# Autodesk Inventor assembly: ClawLauncher
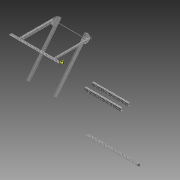
[picture p0: Inventor's stored thumbnail of the model, 180x180]
Saved by Autodesk Inventor 2015 (Build 190159000, 159)
## iProperties
Created: 2016-09-16
Part Number: ClawLauncher
Document SubType Name: Assembly
Designer: wangl
Author: wangl
## Documents named in this file (14)
- M:\StarStuck Prototypes\Prototypes\ClawLauncher.iam
- M:\StarStuck Prototypes\Imported Components\C-Channel 1x2x1x35\C-Channel 1x2x1x35 2.0.ipt
- M:\StarStuck Prototypes\Imported Components\C- Channel 1x2x1x25 2.0\C- Channel 1x2x1x25 2.0.ipt
- M:\StarStuck Prototypes\Imported Components\Chasis Rail 2x1x25\Chasis Rail 2x1x25.ipt
- M:\StarStuck Prototypes\Imported Components\Angle 2x2x35\Angle 2x2x35.ipt
- M:\StarStuck Prototypes\Imported Components\Large Screw .500In\Large Screw .500In.ipt
- M:\StarStuck Prototypes\Imported Components\Flat Bearing\Flat Bearing.ipt
- M:\StarStuck Prototypes\Imported Components\Large Screw .25In\Large Screw .25In.ipt
- M:\StarStuck Prototypes\Imported Components\Regular Nut\Regular Nut.ipt
- M:\StarStuck Prototypes\Imported Components\Axle 12in\Axle 12in.ipt
- M:\StarStuck Prototypes\Imported Components\Shaft Collar\Shaft Collar.ipt
- M:\StarStuck Prototypes\Imported Components\60T HS Gear\60T HS Gear.ipt
- M:\StarStuck Prototypes\Imported Components\HS Gear Metal Insert\HS Gear Metal Insert.ipt
- M:\StarStuck Prototypes\Imported Components\Large 1.00in Screw\Large 1.00in Screw.ipt
## Components (39 placed, 13 different names)
1. C-Channel 1x2x1x35 2.0:1 — Mate:44, Tangent:29, Tangent:30, Tangent:32, Tangent:37
2. C- Channel 1x2x1x25 2.0:1
3. C- Channel 1x2x1x25 2.0:2
4. Chasis Rail 2x1x25:1 — Flush:4, Mate:4, Flush:6, Mate:13, Tangent:13, Tangent:14, Tangent:15, Tangent:16, Mate:16, Mate:17, Mate:23, Mate:24, Tangent:26
5. Chasis Rail 2x1x25:2 — Mate:3, Flush:3, Flush:5, Mate:5, Mate:6, Mate:7, Tangent:7, Tangent:8, Tangent:9, Tangent:10, Mate:14, Mate:15
6. C-Channel 1x2x1x35 2.0:2 — Mate:43, Tangent:33, Tangent:34, Tangent:35, Tangent:36
7. Angle 2x2x35:1
8. Angle 2x2x35:2 — Mate:3, Flush:3, Flush:4, Mate:4, Flush:5, Flush:6, Tangent:1, Tangent:2, Tangent:3, Tangent:4, Mate:18, Mate:19, Mate:20, Mate:21, Tangent:23, Tangent:24, Tangent:25
9. Flat Bearing:1 — Mate:11, Mate:12, Tangent:11, Tangent:12, Mate:13
10. Flat Bearing:2 — Mate:5, Mate:8, Mate:9, Tangent:5, Tangent:6, Insert:1, Insert:3
11. Large Screw .25In:1 — Mate:7, Tangent:1, Tangent:3, Tangent:21
12. Large Screw .25In:2 — Mate:6, Tangent:2, Tangent:4, Tangent:22
13. Large Screw .500In:1 — Mate:8, Tangent:6, Tangent:8, Tangent:10, Tangent:20
14. Large Screw .500In:2 — Mate:9, Tangent:5, Tangent:7, Tangent:9, Tangent:19
15. Large Screw .500In:3 — Mate:12, Tangent:12, Tangent:14, Tangent:15, Tangent:17
16. Large Screw .500In:4 — Mate:11, Tangent:11, Tangent:13, Tangent:16, Tangent:18
17. Regular Nut:1 — Mate:15, Tangent:19
18. Regular Nut:2 — Mate:14, Tangent:20
19. Regular Nut:3 — Mate:16, Tangent:18
20. Regular Nut:4 — Mate:17, Tangent:17
21. Regular Nut:5 — Mate:18, Tangent:21
22. Regular Nut:6 — Mate:19, Tangent:22
23. Regular Nut:7 — Mate:20, Tangent:28
24. Regular Nut:8 — Mate:21, Tangent:27
25. Large Screw .25In:3 — Mate:24, Tangent:23, Tangent:26, Tangent:28
26. Large Screw .25In:4 — Mate:23, Tangent:24, Tangent:25, Tangent:27
27. Axle 12in:1 — Insert:1, Insert:2, Mate:37, Mate:38, Mate:39, Mate:40
28. Shaft Collar:1 — Insert:2, Mate:42
29. Shaft Collar:2 — Insert:3, Mate:41
30. 60T HS Gear:1 — Mate:25, Mate:27, Mate:28, Mate:29, Mate:30, Mate:31, Insert:6, Insert:7, Mate:44
31. 60T HS Gear:2 — Mate:26, Mate:32, Mate:33, Mate:34, Mate:35, Mate:36, Insert:4, Insert:5, Mate:43
32. HS Gear Metal Insert:1 — Mate:26, Mate:33, Mate:35, Mate:39, Mate:40, Mate:41
33. HS Gear Metal Insert:2 — Mate:32, Mate:34, Mate:36
34. HS Gear Metal Insert:3 — Mate:25, Mate:27, Mate:28, Mate:37, Mate:38
35. HS Gear Metal Insert:4 — Mate:29, Mate:30, Mate:31, Mate:42
36. Large 1.00in Screw:1 — Insert:4, Tangent:33, Tangent:36
37. Large 1.00in Screw:2 — Insert:5, Tangent:34, Tangent:35
38. Large 1.00in Screw:3 — Insert:7, Tangent:29, Tangent:32
39. Large 1.00in Screw:4 — Insert:6, Tangent:30, Tangent:37
## Relationships (87: Mate 40, Tangent 36, Insert 7, Flush 4)
- Mate:3: Chasis Rail 2x1x25:2 ↔ Angle 2x2x35:2
- Flush:3: Chasis Rail 2x1x25:2 ↔ Angle 2x2x35:2
- Flush:4: Chasis Rail 2x1x25:1 ↔ Angle 2x2x35:2
- Mate:4: Chasis Rail 2x1x25:1 ↔ Angle 2x2x35:2
- Flush:5: Chasis Rail 2x1x25:2 ↔ Angle 2x2x35:2
- Flush:6: Chasis Rail 2x1x25:1 ↔ Angle 2x2x35:2
- Mate:5: Chasis Rail 2x1x25:2 ↔ Flat Bearing:2
- Mate:6: Chasis Rail 2x1x25:2 ↔ Large Screw .25In:2
- Mate:7: Chasis Rail 2x1x25:2 ↔ Large Screw .25In:1
- Tangent:1: Angle 2x2x35:2 ↔ Large Screw .25In:1
- Tangent:2: Angle 2x2x35:2 ↔ Large Screw .25In:2
- Tangent:3: Angle 2x2x35:2 ↔ Large Screw .25In:1
- Tangent:4: Angle 2x2x35:2 ↔ Large Screw .25In:2
- Mate:8: Flat Bearing:2 ↔ Large Screw .500In:1
- Mate:9: Flat Bearing:2 ↔ Large Screw .500In:2
- Tangent:5: Flat Bearing:2 ↔ Large Screw .500In:2
- Tangent:6: Flat Bearing:2 ↔ Large Screw .500In:1
- Tangent:7: Chasis Rail 2x1x25:2 ↔ Large Screw .500In:2
- Tangent:8: Chasis Rail 2x1x25:2 ↔ Large Screw .500In:1
- Tangent:9: Chasis Rail 2x1x25:2 ↔ Large Screw .500In:2
- Tangent:10: Chasis Rail 2x1x25:2 ↔ Large Screw .500In:1
- Mate:11: Flat Bearing:1 ↔ Large Screw .500In:4
- Mate:12: Flat Bearing:1 ↔ Large Screw .500In:3
- Tangent:11: Flat Bearing:1 ↔ Large Screw .500In:4
- Tangent:12: Flat Bearing:1 ↔ Large Screw .500In:3
- Mate:13: Chasis Rail 2x1x25:1 ↔ Flat Bearing:1
- Tangent:13: Chasis Rail 2x1x25:1 ↔ Large Screw .500In:4
- Tangent:14: Chasis Rail 2x1x25:1 ↔ Large Screw .500In:3
- Tangent:15: Chasis Rail 2x1x25:1 ↔ Large Screw .500In:3
- Tangent:16: Chasis Rail 2x1x25:1 ↔ Large Screw .500In:4
- Mate:14: Chasis Rail 2x1x25:2 ↔ Regular Nut:2
- Mate:15: Chasis Rail 2x1x25:2 ↔ Regular Nut:1
- Mate:16: Chasis Rail 2x1x25:1 ↔ Regular Nut:3
- Mate:17: Chasis Rail 2x1x25:1 ↔ Regular Nut:4
- Tangent:17: Large Screw .500In:3 ↔ Regular Nut:4
- Tangent:18: Large Screw .500In:4 ↔ Regular Nut:3
- Tangent:19: Large Screw .500In:2 ↔ Regular Nut:1
- Tangent:20: Large Screw .500In:1 ↔ Regular Nut:2
- Mate:18: Angle 2x2x35:2 ↔ Regular Nut:5
- Mate:19: Angle 2x2x35:2 ↔ Regular Nut:6
- Mate:20: Angle 2x2x35:2 ↔ Regular Nut:7
- Mate:21: Angle 2x2x35:2 ↔ Regular Nut:8
- Tangent:21: Large Screw .25In:1 ↔ Regular Nut:5
- Tangent:22: Large Screw .25In:2 ↔ Regular Nut:6
- Mate:23: Chasis Rail 2x1x25:1 ↔ Large Screw .25In:4
- Mate:24: Chasis Rail 2x1x25:1 ↔ Large Screw .25In:3
- Tangent:23: Angle 2x2x35:2 ↔ Large Screw .25In:3
- Tangent:24: Angle 2x2x35:2 ↔ Large Screw .25In:4
- Tangent:25: Angle 2x2x35:2 ↔ Large Screw .25In:4
- Tangent:26: Chasis Rail 2x1x25:1 ↔ Large Screw .25In:3
- Tangent:27: Regular Nut:8 ↔ Large Screw .25In:4
- Tangent:28: Regular Nut:7 ↔ Large Screw .25In:3
- Insert:1: Flat Bearing:2 ↔ Axle 12in:1
- Insert:2 (7.62 mm): Axle 12in:1 ↔ Shaft Collar:1
- Insert:3 (7.62 mm): Flat Bearing:2 ↔ Shaft Collar:2
- Mate:25: 60T HS Gear:1 ↔ HS Gear Metal Insert:3
- Mate:26: 60T HS Gear:2 ↔ HS Gear Metal Insert:1
- Mate:27: 60T HS Gear:1 ↔ HS Gear Metal Insert:3
- Mate:28: 60T HS Gear:1 ↔ HS Gear Metal Insert:3
- Mate:29: 60T HS Gear:1 ↔ HS Gear Metal Insert:4
- Mate:30: 60T HS Gear:1 ↔ HS Gear Metal Insert:4
- Mate:31: 60T HS Gear:1 ↔ HS Gear Metal Insert:4
- Mate:32: 60T HS Gear:2 ↔ HS Gear Metal Insert:2
- Mate:33: 60T HS Gear:2 ↔ HS Gear Metal Insert:1
- Mate:34: 60T HS Gear:2 ↔ HS Gear Metal Insert:2
- Mate:35: 60T HS Gear:2 ↔ HS Gear Metal Insert:1
- Mate:36: 60T HS Gear:2 ↔ HS Gear Metal Insert:2
- Mate:37: Axle 12in:1 ↔ HS Gear Metal Insert:3
- Mate:38: Axle 12in:1 ↔ HS Gear Metal Insert:3
- Mate:39: Axle 12in:1 ↔ HS Gear Metal Insert:1
- Mate:40: Axle 12in:1 ↔ HS Gear Metal Insert:1
- Mate:41: Shaft Collar:2 ↔ HS Gear Metal Insert:1
- Mate:42: Shaft Collar:1 ↔ HS Gear Metal Insert:4
- Insert:4: 60T HS Gear:2 ↔ Large 1.00in Screw:1
- Insert:5: 60T HS Gear:2 ↔ Large 1.00in Screw:2
- Insert:6: 60T HS Gear:1 ↔ Large 1.00in Screw:4
- Insert:7: 60T HS Gear:1 ↔ Large 1.00in Screw:3
- Mate:43: C-Channel 1x2x1x35 2.0:2 ↔ 60T HS Gear:2
- Mate:44: C-Channel 1x2x1x35 2.0:1 ↔ 60T HS Gear:1
- Tangent:29: C-Channel 1x2x1x35 2.0:1 ↔ Large 1.00in Screw:3
- Tangent:30: C-Channel 1x2x1x35 2.0:1 ↔ Large 1.00in Screw:4
- Tangent:32: C-Channel 1x2x1x35 2.0:1 ↔ Large 1.00in Screw:3
- Tangent:33: C-Channel 1x2x1x35 2.0:2 ↔ Large 1.00in Screw:1
- Tangent:34: C-Channel 1x2x1x35 2.0:2 ↔ Large 1.00in Screw:2
- Tangent:35: C-Channel 1x2x1x35 2.0:2 ↔ Large 1.00in Screw:2
- Tangent:36: C-Channel 1x2x1x35 2.0:2 ↔ Large 1.00in Screw:1
- Tangent:37: C-Channel 1x2x1x35 2.0:1 ↔ Large 1.00in Screw:4
